# Autodesk Inventor assembly: ASY PNS 1720 bottom FDS1 D1200
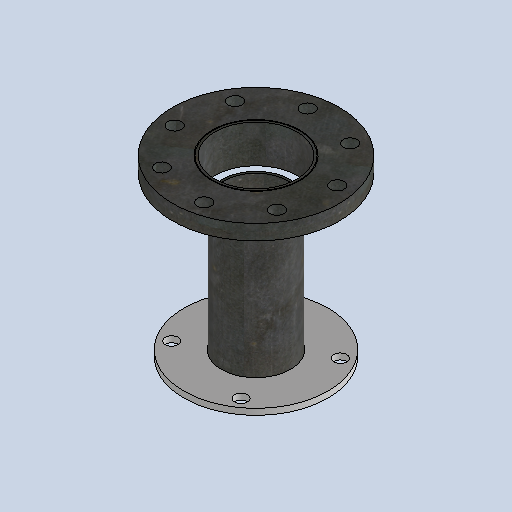
[picture p0: Inventor's stored thumbnail of the model, 512x512]
Saved by Autodesk Inventor 2025.1 (Build 291241020, 241B)
## iProperties
Created: 2025-06-30
Part Number: ASY PNS 1720 bottom FDS1 D1200
Document SubType Name: Assembly
Designer: admin
Author: admin
## Documents named in this file (5)
- C:\Users\user\YandexDisk-badmisterfox\home pc\Inventor\ANP-Antipayuta\ASY PNS 1720 bottom FDS1 D1200.iam
- C:\Users\user\YandexDisk-badmisterfox\home pc\Inventor\ANP-Antipayuta\DIN 2576 Slip-On Flange for Welding Series 1 (ISO) - PN 10 80 x 88.9.ipt
- C:\Users\user\YandexDisk-badmisterfox\home pc\Inventor\ANP-Antipayuta\PNS 1722 FDS  tube 1.ipt
- C:\Users\user\YandexDisk-badmisterfox\home pc\Inventor\ANP-Antipayuta\PNS 1723 FDS tube 2.ipt
- C:\Users\user\YandexDisk-badmisterfox\home pc\Inventor\ANP-Antipayuta\PNS 1721 FDS flange DN90.ipt
## Components (4 placed, 4 different names)
1. DIN 2576 Slip-On Flange for Welding Series 1 (ISO) - PN 10 80 x 88.9.ipt:1
2. PNS 1722 FDS  tube 1.ipt:1 — Rigid:5
3. PNS 1723 FDS tube 2.ipt:1 — Rigid:5
4. PNS 1721 FDS flange DN90.ipt:1
## Relationships (3: WeldJoint 3)
- [WeldJoint]: DIN 2576 Slip-On Flange for Welding Series 1 (ISO) - PN 10 80 x 88.9.ipt:1 ↔ PNS 1722 FDS  tube 1.ipt:1
- [WeldJoint]: PNS 1723 FDS tube 2.ipt:1 ↔ PNS 1721 FDS flange DN90.ipt:1
- Rigid:5 [WeldJoint]: PNS 1722 FDS  tube 1.ipt:1 ↔ PNS 1723 FDS tube 2.ipt:1
